# Autodesk Inventor assembly: Goal Supports
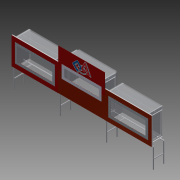
[picture p0: Inventor's stored thumbnail of the model, 180x180]
Saved by Autodesk Inventor 2013 (Build 170138000, 138)
## iProperties
Created: 2013-01-05
Part Number: Goal Supports
Document SubType Name: Assembly
Designer: Phillip
Author: Phillip
## Documents named in this file (6)
- C:\Users\Arpan\Documents\GitHub\frc2013CAD\FIRST Arena 2013\Goal Supports\Goal Supports.iam
- C:\Users\Arpan\Documents\GitHub\frc2013CAD\FIRST Arena 2013\Goal Supports\FE-00103.iam
- C:\Users\Arpan\Documents\GitHub\frc2013CAD\FIRST Arena 2013\Goal Supports\FE-00101.iam
- C:\Users\Arpan\Documents\GitHub\frc2013CAD\FIRST Arena 2013\Goal Supports\FE-00102.iam
- C:\Users\Arpan\Documents\GitHub\frc2013CAD\FIRST Arena 2013\Feeder Goal Station\GE-13028.iam
- C:\Users\Arpan\Documents\GitHub\frc2013CAD\FIRST Arena 2013\Feeder Goal Station\GE-13027.iam
## Components (10 placed, 5 different names)
1. FE-00103:1 [sub-assembly] — Mate:1, Mate:2, Mate:18
2. FE-00101:1 [sub-assembly] — Mate:1, Mate:2, Mate:3, Mate:4, Mate:14, Tangent:3, Tangent:4, Mate:18
3. FE-00102:1 [sub-assembly] — Mate:3, Mate:4, Mate:5, Mate:6, Mate:17
4. FE-00102:2 [sub-assembly] — Mate:7, Mate:8, Mate:9, Mate:10, Mate:20, Mate:21
5. FE-00101:2 [sub-assembly] — Mate:5, Mate:6, Mate:7, Mate:8, Mate:13, Tangent:1, Tangent:2, Mate:17, Mate:20
6. FE-00103:2 [sub-assembly] — Mate:11, Mate:12, Mate:19
7. FE-00101:3 [sub-assembly] — Mate:9, Mate:10, Mate:11, Mate:12, Tangent:5, Tangent:6, Mate:19, Mate:21
8. GE-13028:1 [sub-assembly] — Mate:14, Tangent:3, Tangent:4, Flush:1, Mate:15
9. GE-13028:2 [sub-assembly] — Flush:2, Tangent:5, Tangent:6, Mate:16
10. GE-13027:1 [sub-assembly] — Mate:13, Tangent:1, Tangent:2, Flush:1, Mate:15, Flush:2, Mate:16
## Relationships (29: Mate 21, Tangent 6, Flush 2)
- Mate:1: FE-00103:1 ↔ FE-00101:1
- Mate:2: FE-00103:1 ↔ FE-00101:1
- Mate:3: FE-00101:1 ↔ FE-00102:1
- Mate:4: FE-00101:1 ↔ FE-00102:1
- Mate:5: FE-00102:1 ↔ FE-00101:2
- Mate:6: FE-00102:1 ↔ FE-00101:2
- Mate:7: FE-00102:2 ↔ FE-00101:2
- Mate:8: FE-00102:2 ↔ FE-00101:2
- Mate:9: FE-00102:2 ↔ FE-00101:3
- Mate:10: FE-00102:2 ↔ FE-00101:3
- Mate:11: FE-00103:2 ↔ FE-00101:3
- Mate:12: FE-00103:2 ↔ FE-00101:3
- Mate:13: FE-00101:2 ↔ GE-13027:1
- Tangent:1: FE-00101:2 ↔ GE-13027:1
- Tangent:2: FE-00101:2 ↔ GE-13027:1
- Mate:14: FE-00101:1 ↔ GE-13028:1
- Tangent:3: FE-00101:1 ↔ GE-13028:1
- Tangent:4: FE-00101:1 ↔ GE-13028:1
- Flush:1: GE-13028:1 ↔ GE-13027:1
- Mate:15: GE-13028:1 ↔ GE-13027:1
- Flush:2: GE-13028:2 ↔ GE-13027:1
- Tangent:5: FE-00101:3 ↔ GE-13028:2
- Tangent:6: FE-00101:3 ↔ GE-13028:2
- Mate:16: GE-13028:2 ↔ GE-13027:1
- Mate:17: FE-00102:1 ↔ FE-00101:2
- Mate:18: FE-00103:1 ↔ FE-00101:1
- Mate:19: FE-00103:2 ↔ FE-00101:3
- Mate:20: FE-00102:2 ↔ FE-00101:2
- Mate:21: FE-00102:2 ↔ FE-00101:3
